# Autodesk Inventor assembly: gripper2_v1
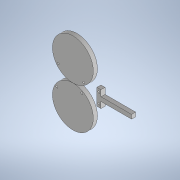
[picture p0: Inventor's stored thumbnail of the model, 180x180]
Saved by Autodesk Inventor 2022 (Build 260153000, 153)
## iProperties
Created: 2022-05-21
Part Number: gripper2_v1
Document SubType Name: Assembly
Designer: kylem
Author: kylem
## Documents named in this file (3)
- C:\Users\kylem\OneDrive\Documents\GitHub\IMML_Contactile_Gripper_Hardware\gripper_v2\gripper2_v1.iam
- C:\Users\kylem\OneDrive\Documents\GitHub\IMML_Contactile_Gripper_Hardware\gripper_v2\drive_shaft.ipt
- C:\Users\kylem\OneDrive\Documents\GitHub\IMML_Contactile_Gripper_Hardware\gripper_v2\drum.ipt
## Components (3 placed, 2 different names)
1. drive_shaft:1 — Mate:1, Mate:2, Flush:1, Flush:2
2. drum:1 — Flush:1, Mate:3, Mate:4
3. drum:2 — Flush:2, Mate:5, Mate:6
## Relationships (8: Mate 6, Flush 2)
- Mate:1: drive_shaft:1
- Mate:2 (-1 mm): drive_shaft:1
- Flush:1: drive_shaft:1 ↔ drum:1
- Mate:3 (10 mm): drum:1
- Mate:4: drum:1
- Flush:2: drive_shaft:1 ↔ drum:2
- Mate:5 (-10 mm): drum:2
- Mate:6: drum:2
